# Autodesk Inventor assembly: Piston Motor Holder assy
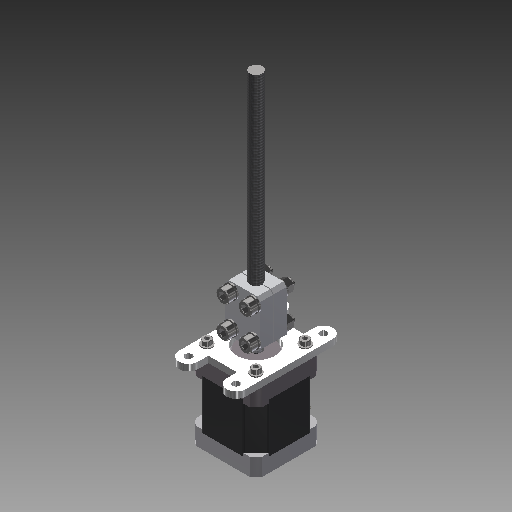
[picture p0: Inventor's stored thumbnail of the model, 512x512]
Saved by Autodesk Inventor 2018 (Build 220112000, 112)
## iProperties
Created: 2017-09-27
Part Number: Piston Motor Holder assy
Document SubType Name: Assembly
Designer: Gabriel Smolnycki
Author: Gabriel Smolnycki
## Documents named in this file (10)
- E:\planb\mechanics\Subassemblies\Piston Motor Holder assy.iam
- E:\planb\mechanics\Electronics\ST4118L1804-A.ipt
- E:\planb\mechanics\Piston\Piston Motor Holder.ipt
- E:\planb\mechanics\Hardware\M3 SS Washer.ipt
- E:\planb\mechanics\Piston\Piston Lead Screw M8.ipt
- E:\planb\mechanics\Piston\Piston Driver Clamp.ipt
- E:\planb\mechanics\Hardware\M4 SS Washer.ipt
- E:\planb\mechanics\Hardware\M4 SS Locknut.ipt
- E:\planb\mechanics\Hardware\M4x25 SS SHCS.ipt
- E:\planb\mechanics\Hardware\M3x8 SS SHCS.ipt
## Components (29 placed, 9 different names)
1. ST4118L1804-A:1 — Insert:1, Insert:2, Insert:11, Insert:12
2. Piston Motor Holder:1 — Insert:1, Insert:2, Insert:3, Insert:4, Insert:5, Insert:6, Flush:1
3. M3 SS Washer:1 — Insert:6
4. M3 SS Washer:2 — Insert:3
5. M3 SS Washer:3 — Insert:4
6. M3 SS Washer:4 — Insert:5
7. M3x8 SS SHCS:1
8. M3x8 SS SHCS:2
9. M3x8 SS SHCS:3
10. M3x8 SS SHCS:4
11. Piston Lead Screw M8:1 — Insert:13
12. Piston Driver Clamp:1 — Insert:11, Flush:1, Mate:1, Insert:13, Insert:18, Insert:19, Insert:20, Insert:21
13. Piston Driver Clamp:2 — Insert:12, Mate:1, Insert:14, Insert:15, Insert:16, Insert:17
14. M4 SS Washer:1 — Insert:20, Insert:29
15. M4 SS Washer:2 — Insert:21, Insert:28
16. M4 SS Washer:3 — Insert:16
17. M4 SS Washer:4 — Insert:14
18. M4 SS Washer:5 — Insert:15
19. M4 SS Washer:6 — Insert:17
20. M4 SS Washer:7 — Insert:19, Insert:27
21. M4 SS Washer:8 — Insert:18, Insert:23
22. M4 SS Locknut:1 — Insert:23
23. M4 SS Locknut:2 — Insert:28
24. M4 SS Locknut:3 — Insert:27
25. M4 SS Locknut:4 — Insert:29
26. M4x25 SS SHCS:1
27. M4x25 SS SHCS:2
28. M4x25 SS SHCS:3
29. M4x25 SS SHCS:4
## Relationships (31: Insert 29, Flush 1, Mate 1)
- Insert:1: ST4118L1804-A:1 ↔ Piston Motor Holder:1
- Insert:2: ST4118L1804-A:1 ↔ Piston Motor Holder:1
- Insert:3: Piston Motor Holder:1 ↔ M3 SS Washer:2
- Insert:4: Piston Motor Holder:1 ↔ M3 SS Washer:3
- Insert:5: Piston Motor Holder:1 ↔ M3 SS Washer:4
- Insert:6: Piston Motor Holder:1 ↔ M3 SS Washer:1
- [Insert]: M3 SS Washer:2 ↔ M3x8 SS SHCS:4
- [Insert]: M3 SS Washer:3 ↔ M3x8 SS SHCS:3
- [Insert]: M3 SS Washer:4 ↔ M3x8 SS SHCS:2
- [Insert]: M3 SS Washer:1 ↔ M3x8 SS SHCS:1
- Insert:11: ST4118L1804-A:1 ↔ Piston Driver Clamp:1
- Flush:1: Piston Motor Holder:1 ↔ Piston Driver Clamp:1
- Insert:12: ST4118L1804-A:1 ↔ Piston Driver Clamp:2
- Mate:1: Piston Driver Clamp:1 ↔ Piston Driver Clamp:2
- Insert:13: Piston Lead Screw M8:1 ↔ Piston Driver Clamp:1
- Insert:14: Piston Driver Clamp:2 ↔ M4 SS Washer:4
- Insert:15: Piston Driver Clamp:2 ↔ M4 SS Washer:5
- Insert:16: Piston Driver Clamp:2 ↔ M4 SS Washer:3
- Insert:17: Piston Driver Clamp:2 ↔ M4 SS Washer:6
- Insert:18: Piston Driver Clamp:1 ↔ M4 SS Washer:8
- Insert:19: Piston Driver Clamp:1 ↔ M4 SS Washer:7
- Insert:20: Piston Driver Clamp:1 ↔ M4 SS Washer:1
- Insert:21: Piston Driver Clamp:1 ↔ M4 SS Washer:2
- [Insert]: M4 SS Washer:5 ↔ M4x25 SS SHCS:4
- Insert:23: M4 SS Washer:8 ↔ M4 SS Locknut:1
- [Insert]: M4 SS Washer:4 ↔ M4x25 SS SHCS:3
- [Insert]: M4 SS Washer:6 ↔ M4x25 SS SHCS:2
- [Insert]: M4 SS Washer:3 ↔ M4x25 SS SHCS:1
- Insert:27: M4 SS Washer:7 ↔ M4 SS Locknut:3
- Insert:28: M4 SS Washer:2 ↔ M4 SS Locknut:2
- Insert:29: M4 SS Washer:1 ↔ M4 SS Locknut:4
